# Autodesk Inventor assembly: Ensamble
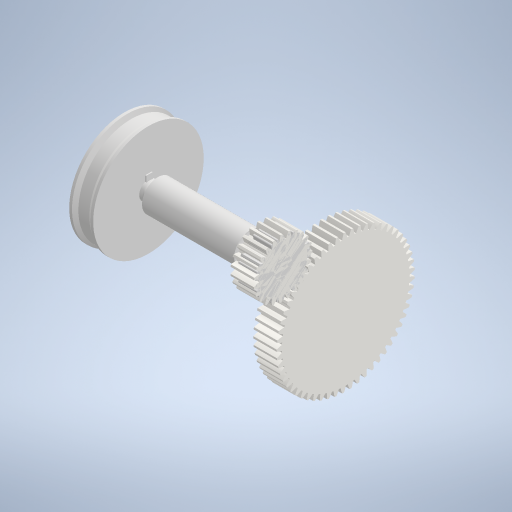
[picture p0: Inventor's stored thumbnail of the model, 512x512]
Saved by Autodesk Inventor 2024 (Build 280153000, 153)
## iProperties
Created: 2024-03-20
Part Number: Ensamble
Document SubType Name: Assembly
Designer: USUARIO
Author: USUARIO
## Documents named in this file (6)
- C:\Users\USUARIO\Documents\2024\UNIVERSIDAD\DINAMICA\LAB\Ensamble.iam
- C:\Users\USUARIO\Downloads\EJE_CUÑEROS.ipt
- C:\Users\USUARIO\Downloads\ENGRANE.ipt
- C:\Users\USUARIO\Downloads\POLEA.ipt
- C:\Users\USUARIO\Downloads\CUÑA.ipt
- C:\Users\USUARIO\Documents\2024\UNIVERSIDAD\DINAMICA\LAB\Assembly1\Design Accelerator\Spur Gears1.iam
## Components (6 placed, 5 different names)
1. EJE_CUÑEROS:1 — Rotational:1, Flush:1, Mate:1, Rigid:1, Rotational:2, Flush:2, Mate:2, Rigid:2, Flush:3
2. ENGRANE:1 — Rotational:2, Flush:2, Mate:2, Rotational:3, Flush:3
3. POLEA:1 — Rotational:1, Flush:1, Mate:1
4. CUÑA:1 — Rigid:1
5. Spur Gears:1 [sub-assembly] — Rotational:3
6. CUÑA:2 — Rigid:2
## Relationships (10: RevoluteJoint 3, Flush 3, Mate 2, WeldJoint 2)
- Rotational:1 [RevoluteJoint]: EJE_CUÑEROS:1 ↔ POLEA:1
- Flush:1: EJE_CUÑEROS:1 ↔ POLEA:1
- Mate:1: EJE_CUÑEROS:1 ↔ POLEA:1
- Rigid:1 [WeldJoint]: EJE_CUÑEROS:1 ↔ CUÑA:1
- Rotational:2 [RevoluteJoint]: EJE_CUÑEROS:1 ↔ ENGRANE:1
- Flush:2: EJE_CUÑEROS:1 ↔ ENGRANE:1
- Mate:2: EJE_CUÑEROS:1 ↔ ENGRANE:1
- Rigid:2 [WeldJoint]: EJE_CUÑEROS:1 ↔ CUÑA:2
- Rotational:3 [RevoluteJoint]: ENGRANE:1 ↔ Spur Gears:1
- Flush:3: EJE_CUÑEROS:1 ↔ ENGRANE:1
